# Autodesk Inventor assembly: 000.400 - Рычаг 2
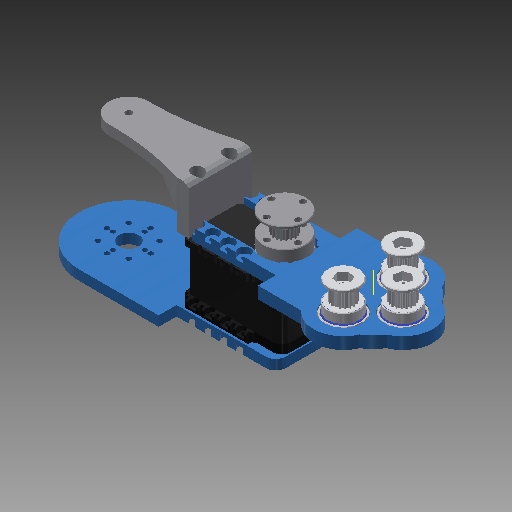
[picture p0: Inventor's stored thumbnail of the model, 512x512]
Saved by Autodesk Inventor 2019 (Build 230136000, 136)
## iProperties
Created: 2020-03-18
Part Number: 000.400 - Рычаг 2
Material: Типовые
Document SubType Name: Assembly
Designer: Петров Иван
Author: Петров Иван
## Documents named in this file (9)
- E:\IVAN\Ivan_desktop\Kvantorium\Competitions\INOP_2020\hardware\SCARA(Dynamixels)\000.400 - Рычаг 2.iam
- E:\IVAN\Ivan_desktop\Kvantorium\Competitions\INOP_2020\hardware\SCARA(Dynamixels)\000.401 - Опорная платформа.ipt
- E:\IVAN\Ivan_desktop\Kvantorium\Competitions\INOP_2020\hardware\SCARA(Dynamixels)\components\Сервомотор Dynamixel AX-12-A\AX-12A.iam
- E:\IVAN\Ivan_desktop\Kvantorium\Competitions\INOP_2020\hardware\SCARA(Dynamixels)\000.402 - Опорная платформа верхняя.ipt
- E:\IVAN\Ivan_desktop\Kvantorium\Competitions\INOP_2020\hardware\SCARA(Dynamixels)\components\Подшипник 626Z.ipt
- E:\IVAN\Ivan_desktop\Kvantorium\Competitions\INOP_2020\hardware\SCARA(Dynamixels)\components\Timing Pulley 18T.ipt
- E:\IVAN\Ivan_desktop\Kvantorium\Competitions\INOP_2020\hardware\SCARA(Dynamixels)\components\Сервомотор Dynamixel AX-12-A\AX-12A-04.ipt
- E:\IVAN\Ivan_desktop\Kvantorium\Competitions\INOP_2020\hardware\SCARA(Dynamixels)\000.400 - Рычаг 2\000.404 - Проставка шкива.ipt
- E:\IVAN\Ivan_desktop\Kvantorium\Competitions\INOP_2020\hardware\SCARA(Dynamixels)\000.403 - Верхний рычаг.ipt
## Components (12 placed, 8 different names)
1. 000.401 - Опорная платформа:1 — Совмещение:1, Совмещение:2, Совмещение:3, Совмещение:24
2. AX-12A:1 [sub-assembly] — Совмещение:1, Совмещение:2, Совмещение:3, Совмещение:4, Совмещение:5, Совмещение:17, Совмещение:18, Совмещение:26, Совмещение:27, Совмещение:28
3. 000.402 - Опорная платформа верхняя:1 — Совмещение:4, Совмещение:5, Заподлицо:8, Совмещение:8, Совмещение:9, Заподлицо:9, Заподлицо:10, Совмещение:10, Совмещение:26
4. Подшипник 626Z:1 — Заподлицо:10, Совмещение:10, Совмещение:11, Совмещение:14
5. Подшипник 626Z:2 — Совмещение:9, Заподлицо:9, Совмещение:12, Совмещение:16
6. Подшипник 626Z:3 — Заподлицо:8, Совмещение:8, Совмещение:13, Совмещение:15
7. Timing Pulley 18T:1 — Совмещение:11, Совмещение:14, Направление навивки:2
8. Timing Pulley 18T:2 — Совмещение:13, Совмещение:15, Направление навивки:1, Направление навивки:3
9. Timing Pulley 18T:3 — Совмещение:12, Совмещение:16, Направление навивки:1, Направление навивки:2
10. AX-12A-04:1 — Совмещение:17, Совмещение:18, Направление навивки:3, Заподлицо:11, Совмещение:21, Совмещение:22
11. 000.404 - Проставка шкива:1 — Заподлицо:11, Совмещение:21, Совмещение:22
12. 000.403 - Верхний рычаг:1 — Совмещение:24, Совмещение:27, Совмещение:28
## Relationships (29: Mate 22, Flush 4, RelateRotation 3)
- Совмещение:1 [Mate]: 000.401 - Опорная платформа:1 ↔ AX-12A:1
- Совмещение:2 [Mate]: 000.401 - Опорная платформа:1 ↔ AX-12A:1
- Совмещение:3 [Mate]: 000.401 - Опорная платформа:1 ↔ AX-12A:1
- Совмещение:4 [Mate]: AX-12A:1 ↔ 000.402 - Опорная платформа верхняя:1
- Совмещение:5 [Mate]: AX-12A:1 ↔ 000.402 - Опорная платформа верхняя:1
- Заподлицо:8 [Flush]: 000.402 - Опорная платформа верхняя:1 ↔ Подшипник 626Z:3
- Совмещение:8 [Mate]: 000.402 - Опорная платформа верхняя:1 ↔ Подшипник 626Z:3
- Совмещение:9 [Mate]: 000.402 - Опорная платформа верхняя:1 ↔ Подшипник 626Z:2
- Заподлицо:9 [Flush]: 000.402 - Опорная платформа верхняя:1 ↔ Подшипник 626Z:2
- Заподлицо:10 [Flush]: 000.402 - Опорная платформа верхняя:1 ↔ Подшипник 626Z:1
- Совмещение:10 [Mate]: 000.402 - Опорная платформа верхняя:1 ↔ Подшипник 626Z:1
- Совмещение:11 [Mate]: Подшипник 626Z:1 ↔ Timing Pulley 18T:1
- Совмещение:12 [Mate]: Подшипник 626Z:2 ↔ Timing Pulley 18T:3
- Совмещение:13 [Mate]: Подшипник 626Z:3 ↔ Timing Pulley 18T:2
- Совмещение:14 [Mate]: Подшипник 626Z:1 ↔ Timing Pulley 18T:1
- Совмещение:15 [Mate]: Подшипник 626Z:3 ↔ Timing Pulley 18T:2
- Совмещение:16 [Mate]: Подшипник 626Z:2 ↔ Timing Pulley 18T:3
- Направление навивки:1 [RelateRotation] (1 ul): Timing Pulley 18T:2 ↔ Timing Pulley 18T:3
- Направление навивки:2 [RelateRotation] (1 ul): Timing Pulley 18T:1 ↔ Timing Pulley 18T:3
- Совмещение:17 [Mate]: AX-12A:1 ↔ AX-12A-04:1
- Совмещение:18 [Mate]: AX-12A:1 ↔ AX-12A-04:1
- Направление навивки:3 [RelateRotation] (1 ul): Timing Pulley 18T:2 ↔ AX-12A-04:1
- Заподлицо:11 [Flush]: AX-12A-04:1 ↔ 000.404 - Проставка шкива:1
- Совмещение:21 [Mate]: AX-12A-04:1 ↔ 000.404 - Проставка шкива:1
- Совмещение:22 [Mate]: AX-12A-04:1 ↔ 000.404 - Проставка шкива:1
- Совмещение:24 [Mate]: 000.401 - Опорная платформа:1 ↔ 000.403 - Верхний рычаг:1
- Совмещение:26 [Mate]: AX-12A:1 ↔ 000.402 - Опорная платформа верхняя:1
- Совмещение:27 [Mate]: AX-12A:1 ↔ 000.403 - Верхний рычаг:1
- Совмещение:28 [Mate]: AX-12A:1 ↔ 000.403 - Верхний рычаг:1
